# Autodesk Inventor assembly: Final box
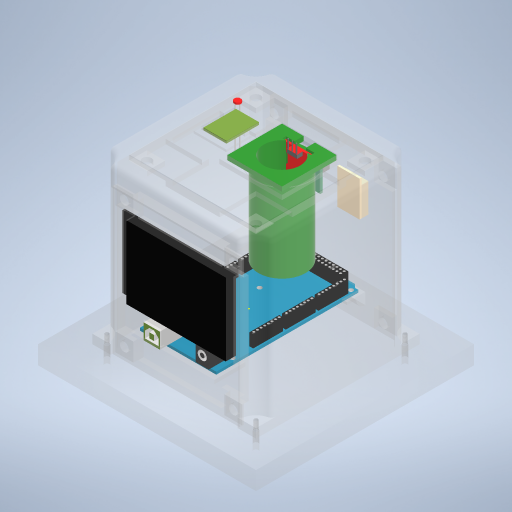
[picture p0: Inventor's stored thumbnail of the model, 512x512]
Saved by Autodesk Inventor 2023 (Build 270158000, 158)
## iProperties
Created: 2023-09-21
Part Number: Final box
Document SubType Name: Assembly
Designer: Gage
Author: Gage
## Documents named in this file (6)
- C:\Users\Gage\OneDrive\Desktop\Autodesk Inventor\207\Final box.iam
- C:\Users\Gage\OneDrive\Desktop\Autodesk Inventor\207\Eg207FinalProjectBox.ipt
- C:\Users\Gage\OneDrive\Desktop\Autodesk Inventor\207\BasePlate.ipt
- C:\Users\Gage\OneDrive\Desktop\Autodesk Inventor\207\front pannel.iam
- C:\Users\Gage\OneDrive\Desktop\Autodesk Inventor\207\Top Plate.iam
- C:\Users\Gage\OneDrive\Desktop\Autodesk Inventor\207\BackPlate.iam
## Components (5 placed, 5 different names)
1. Eg207FinalProjectBox:1 — Mate:19, Mate:20, Mate:33, Mate:34, Mate:35, Mate:36
2. BasePlate:1 — Mate:19, Mate:20
3. front pannel:1 [sub-assembly] — Mate:33
4. Top Plate:1 [sub-assembly] — Mate:34
5. BackPlate:1 [sub-assembly] — Mate:35, Mate:36
## Relationships (6: Mate 6)
- Mate:19: Eg207FinalProjectBox:1 ↔ BasePlate:1
- Mate:20: Eg207FinalProjectBox:1 ↔ BasePlate:1
- Mate:33: Eg207FinalProjectBox:1 ↔ front pannel:1
- Mate:34: Eg207FinalProjectBox:1 ↔ Top Plate:1
- Mate:35: Eg207FinalProjectBox:1 ↔ BackPlate:1
- Mate:36: Eg207FinalProjectBox:1 ↔ BackPlate:1
